# Autodesk Inventor assembly: tentioner1
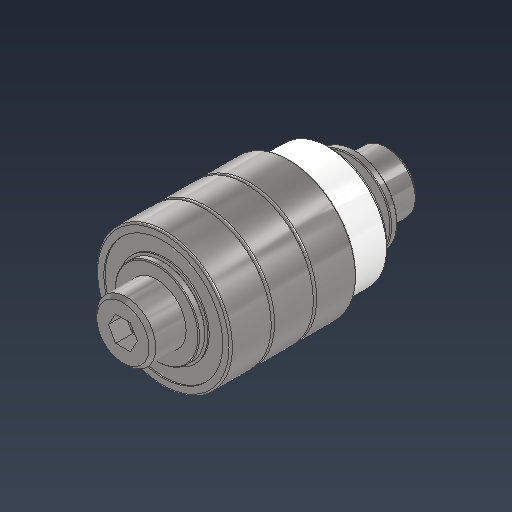
[picture p0: Inventor's stored thumbnail of the model, 512x512]
Saved by Autodesk Inventor 2021 (Build 250183000, 183)
## iProperties
Created: 2021-07-18
Part Number: tentioner1
Document SubType Name: Assembly
Designer: yuta0
Mass: 26.9565 g
Surface Area: 38.6954 cm^2
Volume: 3.73485 cm^3
Density: 7.21757 g/cm^3
Author: yuta0
## Documents named in this file (6)
- C:\Users\yuta0\Desktop\catchrobo_robot\tentioner1.iam
- C:\Users\yuta0\Desktop\catchrobo_robot\base19.ipt
- C:\Users\yuta0\Desktop\catchrobo_robot\ARF-420E.ipt
- C:\Users\yuta0\Desktop\catchrobo_robot\B688ZZ.ipt
- C:\Users\yuta0\Desktop\catchrobo_robot\CB4-5.ipt
- C:\Users\yuta0\Desktop\catchrobo_robot\WSJ-STN-M4.ipt
## Components (9 placed, 5 different names)
1. spacer3:1 — フラッシュ:1, メイト:2
2. unir-spacer4:1 — フラッシュ:1, メイト:1, メイト:3, メイト:7, メイト:8, メイト:13
3. CB4-5:1 — メイト:3, メイト:11, メイト:12
4. CB4-5:2 — メイト:9, メイト:10
5. WSJ-STN-M4:1 — メイト:7, メイト:8, メイト:9, メイト:10
6. WSJ-STN-M4:2 — メイト:11, メイト:12, メイト:13
7. B688ZZ:1 — メイト:1, メイト:2
8. B688ZZ:2
9. B688ZZ:3
## Component patterns: (3 elements, first: B688ZZ:1)
## Relationships (11: Mate 10, Flush 1)
- フラッシュ:1 [Flush]: spacer3:1 ↔ unir-spacer4:1
- メイト:1 [Mate]: unir-spacer4:1 ↔ B688ZZ:1
- メイト:2 [Mate]: spacer3:1 ↔ B688ZZ:1
- メイト:3 [Mate]: unir-spacer4:1 ↔ CB4-5:1
- メイト:7 [Mate]: unir-spacer4:1 ↔ WSJ-STN-M4:1
- メイト:8 [Mate]: unir-spacer4:1 ↔ WSJ-STN-M4:1
- メイト:9 [Mate]: CB4-5:2 ↔ WSJ-STN-M4:1
- メイト:10 [Mate]: CB4-5:2 ↔ WSJ-STN-M4:1
- メイト:11 [Mate]: CB4-5:1 ↔ WSJ-STN-M4:2
- メイト:12 [Mate]: CB4-5:1 ↔ WSJ-STN-M4:2
- メイト:13 [Mate] (2 mm): unir-spacer4:1 ↔ WSJ-STN-M4:2
